# Autodesk Inventor assembly: !intake
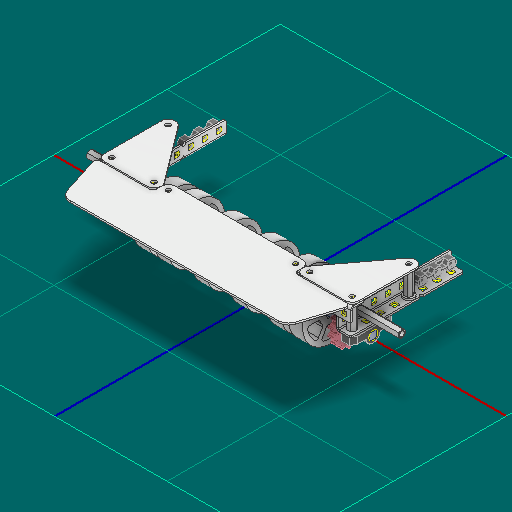
[picture p0: Inventor's stored thumbnail of the model, 512x512]
Saved by Autodesk Inventor 2025 (Build 290162000, 162)
## iProperties
Created: 2024-07-02
Part Number: !intake
Document SubType Name: Assembly
Designer: Averey Ku
Author: Averey Ku
## Documents named in this file (13)
- C:\Users\avere\vex_robotics_high_stakes\hardware\cad\EARLY_SEASON\intake\!intake.iam
- C:\Users\avere\vex_robotics_high_stakes\hardware\cad\VEX-CAD-Inventor\Structure\Angle\Aluminum 1x1\Alu Angle 1x1x8.ipt
- C:\Users\avere\vex_robotics_high_stakes\hardware\cad\VEX-CAD-Inventor\Structure\Standoff\Standoff 1.50.ipt
- D:\vex_robotics_high_stakes\hardware\cad\VEX-CAD-Inventor\Structure\Standoff.ipt
- C:\Users\avere\vex_robotics_high_stakes\hardware\cad\VEX-CAD-Inventor\Structure\Standoff\Standoff .875.ipt
- C:\Users\avere\vex_robotics_high_stakes\hardware\cad\EARLY_SEASON\intake\custom_parts\intake_gusset.ipt
- C:\Users\avere\vex_robotics_high_stakes\hardware\cad\VEX-CAD-Inventor\Motion\Spacers\Washer Teflon\TWasher .375 OD x .06250.ipt
- D:\vex_robotics_high_stakes\hardware\cad\VEX-CAD-Inventor\Motion\Spacers\Washer Teflon.ipt
- C:\Users\avere\vex_robotics_high_stakes\hardware\cad\EARLY_SEASON\intake\custom_parts\intake_wedge.ipt
- C:\Users\avere\vex_robotics_high_stakes\hardware\cad\VEX-CAD-Inventor\Motion\Shaft HS\HS Pillow Bearing Block.ipt
- C:\Users\avere\vex_robotics_high_stakes\hardware\cad\VEX-CAD-Inventor\Structure\Angle\Aluminum 1x1\Alu Angle 1x1x18.ipt
- C:\Users\avere\vex_robotics_high_stakes\hardware\cad\VEX-CAD-Inventor\Motion\Shaft LS\Bearing Flat Low Profile.ipt
- C:\Users\avere\vex_robotics_high_stakes\hardware\cad\EARLY_SEASON\intake\roller.iam
## Components (19 placed, 10 different names)
1. Alu Angle 1x1x8:1 — Insert:10, Insert:14, Mate:7, Insert:20, Mate:12
2. Standoff 1.50:1
3. Standoff .875:2 — Insert:16
4. Alu Angle 1x1x8:2 — Insert:8, Insert:11, Insert:13, Mate:6, Insert:19, Mate:11
5. Standoff .875:3 — Insert:15
6. intake_gusset:1 — Mate:8, Insert:22
7. intake_gusset:2 — Insert:18, Mate:10
8. Standoff .875:4 — Insert:7
9. TWasher .375 OD x .06250:1 — Insert:7, Insert:8
10. TWasher .375 OD x .06250:2 — Insert:9, Insert:10
11. Standoff .875:5 — Insert:9
12. Standoff 1.50:6 — Insert:11
13. intake_wedge:1 — Insert:17, Mate:9
14. HS Pillow Bearing Block:1 — Insert:13, Mate:6
15. HS Pillow Bearing Block:2 — Insert:14, Mate:7, Insert:21
16. Alu Angle 1x1x18:1 — Insert:15, Mate:8, Insert:16, Insert:17, Mate:9, Insert:18, Mate:10, Insert:22
17. Bearing Flat Low Profile:1 — Insert:19, Mate:11
18. Bearing Flat Low Profile:2 — Insert:20, Mate:12
19. roller:1 [sub-assembly] — Insert:21
## Relationships (26: Insert 18, Mate 8)
- [Insert]: Alu Angle 1x1x8:1 ↔ Standoff 1.50:1
- [Insert]: Alu Angle 1x1x8:1 ↔ Standoff .875:2
- [Insert]: Alu Angle 1x1x8:2 ↔ Standoff .875:3
- [Mate]: Alu Angle 1x1x8:1 ↔ Alu Angle 1x1x8:2
- Insert:7: Standoff .875:4 ↔ TWasher .375 OD x .06250:1
- Insert:8: Alu Angle 1x1x8:2 ↔ TWasher .375 OD x .06250:1
- Insert:9: TWasher .375 OD x .06250:2 ↔ Standoff .875:5
- Insert:10: Alu Angle 1x1x8:1 ↔ TWasher .375 OD x .06250:2
- Insert:11: Alu Angle 1x1x8:2 ↔ Standoff 1.50:6
- Insert:13: Alu Angle 1x1x8:2 ↔ HS Pillow Bearing Block:1
- Mate:6: Alu Angle 1x1x8:2 ↔ HS Pillow Bearing Block:1
- Insert:14: Alu Angle 1x1x8:1 ↔ HS Pillow Bearing Block:2
- Mate:7: Alu Angle 1x1x8:1 ↔ HS Pillow Bearing Block:2
- Insert:15: Standoff .875:3 ↔ Alu Angle 1x1x18:1
- Mate:8: intake_gusset:1 ↔ Alu Angle 1x1x18:1
- Insert:16: Standoff .875:2 ↔ Alu Angle 1x1x18:1
- Insert:17: intake_wedge:1 ↔ Alu Angle 1x1x18:1
- Mate:9: intake_wedge:1 ↔ Alu Angle 1x1x18:1
- Insert:18: intake_gusset:2 ↔ Alu Angle 1x1x18:1
- Mate:10: intake_gusset:2 ↔ Alu Angle 1x1x18:1
- Insert:19: Alu Angle 1x1x8:2 ↔ Bearing Flat Low Profile:1
- Mate:11: Alu Angle 1x1x8:2 ↔ Bearing Flat Low Profile:1
- Insert:20: Alu Angle 1x1x8:1 ↔ Bearing Flat Low Profile:2
- Mate:12: Alu Angle 1x1x8:1 ↔ Bearing Flat Low Profile:2
- Insert:21: HS Pillow Bearing Block:2 ↔ roller:1
- Insert:22: intake_gusset:1 ↔ Alu Angle 1x1x18:1
